# Autodesk Inventor assembly: naswietlarka uv
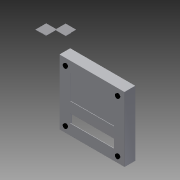
[picture p0: Inventor's stored thumbnail of the model, 180x180]
Saved by Autodesk Inventor 2014 (Build 180170000, 170)
## iProperties
Created: 2013-08-20
Part Number: naswietlarka uv
Document SubType Name: Assembly
Designer: Kisieel
Author: Kisieel
## Documents named in this file (23)
- D:\szkola\synergia\Naswietlarka\naswietlarka uv.iam
- D:\szkola\synergia\Naswietlarka\szyba.ipt
- D:\szkola\synergia\Naswietlarka\kątownik 1.ipt
- D:\szkola\synergia\Naswietlarka\kątownik 2.ipt
- D:\szkola\synergia\Naswietlarka\kątownik 3.ipt
- D:\szkola\synergia\Naswietlarka\blacha1.ipt
- D:\szkola\synergia\Naswietlarka\blacha2.ipt
- D:\szkola\synergia\Naswietlarka\kątownik_mały1.ipt
- D:\szkola\synergia\Naswietlarka\kątownik_mały2.ipt
- D:\szkola\synergia\Naswietlarka\kątownik_mały3.ipt
- D:\szkola\synergia\Naswietlarka\nóżka.ipt
- D:\szkola\synergia\Naswietlarka\świetlówka.ipt
- D:\szkola\synergia\Naswietlarka\uchwytG5.ipt
- D:\szkola\synergia\Naswietlarka\uchwytG5_MIR.ipt
- D:\szkola\synergia\Naswietlarka\Część5.ipt
- D:\szkola\synergia\Naswietlarka\wozek.ipt
- D:\szkola\synergia\Naswietlarka\podpora.ipt
- D:\szkola\synergia\Naswietlarka\kątownik_bloczek.ipt
- D:\szkola\synergia\Naswietlarka\poprzeczka.ipt
- D:\szkola\synergia\Naswietlarka\bloczek.ipt
- D:\szkola\synergia\Naswietlarka\sworzeń.ipt
- D:\szkola\synergia\Naswietlarka\zawias.ipt
- D:\szkola\synergia\Naswietlarka\zawias2.ipt
## Components (40 placed, 22 different names)
1. szyba:1 — Zestawiający:2, Równoległy:1, Zestawiający:3, Równoległy:2, Zestawiający:4, Zestawiający:6, Zestawiający:22
2. kątownik 1:1 — Zestawiający:2, Równoległy:1, Równoległy:3, Zestawiający:7, Równoległy:7, Równoległy:8, Zestawiający:10, Zestawiający:16, Zestawiający:24, Równoległy:14, Zestawiający:27, Styczny:2, Zestawiający:29, Styczny:5, Równoległy:19, Równoległy:21
3. kątownik 1:2 — Zestawiający:3, Równoległy:2, Równoległy:3, Równoległy:4, Równoległy:5, Zestawiający:5, Równoległy:6, Zestawiający:11, Zestawiający:15, Zestawiający:20, Zestawiający:23, Równoległy:13, Zestawiający:28, Styczny:4, Styczny:8, Zestawiający:33
4. kątownik 2:1 — Zestawiający:4, Równoległy:4, Równoległy:5, Zestawiający:8, Zestawiający:14, Równoległy:9, Styczny:1, Styczny:3, Zestawiający:72, Zestawiający:74
5. kątownik 3:1 — Zestawiający:5, Zestawiający:6, Równoległy:6, Zestawiający:9, Zestawiający:18, Zestawiający:25, Zestawiający:58, Zestawiający:62
6. kątownik 2:2 — Zestawiający:7, Równoległy:7, Równoległy:8, Zestawiający:26, Styczny:6, Zestawiający:30, Styczny:7, Zestawiający:32, Zestawiający:34
7. blacha1:1 — Zestawiający:8, Zestawiający:9, Zestawiający:10, Zestawiający:61, Zestawiający:73, Zestawiający:76
8. blacha2:1 — Zestawiający:11, Zestawiający:33, Zestawiający:34
9. kątownik_mały1:1 — Zestawiający:14, Równoległy:9, Zestawiający:15, Równoległy:10, Zestawiający:17
10. kątownik_mały2:1 — Zestawiający:16, Równoległy:10, Zestawiający:17, Równoległy:11, Zestawiający:19
11. kątownik_mały1:2 — Zestawiający:18, Równoległy:11, Zestawiający:19, Równoległy:12, Zestawiający:21, Zestawiający:22
12. kątownik_mały2:2 — Zestawiający:20, Równoległy:12, Zestawiający:21
13. kątownik_mały3:1 — Zestawiający:23, Równoległy:13, Zestawiający:26
14. kątownik_mały3:2 — Zestawiający:24, Równoległy:14, Zestawiający:25
15. nóżka:1 — Zestawiający:27, Styczny:1, Styczny:2, Zestawiający:31
16. nóżka:2 — Zestawiający:28, Styczny:3, Styczny:4
17. nóżka:3 — Zestawiający:30, Styczny:7, Styczny:8
18. nóżka:4 — Zestawiający:29, Styczny:5, Styczny:6
19. Część5:1 — Zestawiający:52, Zestawiający:53, Zestawiający:58, Symetria:1
20. wozek:1 — Zestawiający:52, Zestawiający:53, Zestawiający:57, Równoległy:15, Równoległy:16
21. Część5:2 — Zestawiający:61, Zestawiający:62, Zestawiający:69, Symetria:1
22. wozek:2 — Zestawiający:63, Równoległy:17, Zestawiający:64, Zestawiający:69, Zestawiający:78
23. podpora:1 — Zestawiający:57, Równoległy:15, Równoległy:16, Zestawiający:70, Równoległy:20, Zestawiający:71
24. podpora:2 — Zestawiający:63, Równoległy:17, Zestawiający:64, Zestawiający:65, Zestawiający:66, Równoległy:18, Zestawiający:77, Równoległy:22
25. kątownik_bloczek:1 — Zestawiający:72, Zestawiający:73, Zestawiający:75, Symetria:2, Zestawiający:79, Obrotowe:1
26. kątownik_bloczek:2 — Zestawiający:74, Zestawiający:75, Zestawiający:76, Symetria:2, Zestawiający:81
27. poprzeczka:1 — Zestawiający:77, Równoległy:22, Zestawiający:78
28. bloczek:1 — Zestawiający:80, Zestawiający:81
29. sworzeń:1 — Zestawiający:79, Obrotowe:1, Zestawiający:80
30. zawias:1
31. zawias2:1
32. świetlówka:1 — Zestawiający:35, Zestawiający:36, Zestawiający:37, Zestawiający:38, Kąt:2, Kąt:3
33. uchwytG5:1 — Zestawiający:35, Zestawiający:38, Kąt:1, Kąt:3, Równoległy:18
34. uchwytG5_MIR:1 — Zestawiający:36, Zestawiający:37, Kąt:1, Kąt:2
35. świetlówka:2
36. uchwytG5:2
37. uchwytG5_MIR:2
38. świetlówka:3
39. uchwytG5:3 — Zestawiający:65, Zestawiający:66
40. uchwytG5_MIR:3 — Zestawiający:70, Równoległy:20, Zestawiający:71
## Component patterns: (3 elements, first: świetlówka:1 + uchwytG5:1 + uchwytG5_MIR:1)
## Relationships (95: Mate 59, Flush 22, Tangent 8, Angle 3, Symmetry 2, RevoluteJoint 1)
- Zestawiający:2 [Mate]: szyba:1 ↔ kątownik 1:1
- Równoległy:1 [Flush]: szyba:1 ↔ kątownik 1:1
- Zestawiający:3 [Mate]: szyba:1 ↔ kątownik 1:2
- Równoległy:2 [Flush]: szyba:1 ↔ kątownik 1:2
- Równoległy:3 [Flush]: kątownik 1:1 ↔ kątownik 1:2
- Zestawiający:4 [Mate]: szyba:1 ↔ kątownik 2:1
- Równoległy:4 [Flush]: kątownik 1:2 ↔ kątownik 2:1
- Równoległy:5 [Flush]: kątownik 1:2 ↔ kątownik 2:1
- Zestawiający:5 [Mate]: kątownik 1:2 ↔ kątownik 3:1
- Zestawiający:6 [Mate]: szyba:1 ↔ kątownik 3:1
- Równoległy:6 [Flush]: kątownik 1:2 ↔ kątownik 3:1
- Zestawiający:7 [Mate]: kątownik 1:1 ↔ kątownik 2:2
- Równoległy:7 [Flush]: kątownik 1:1 ↔ kątownik 2:2
- Równoległy:8 [Flush]: kątownik 1:1 ↔ kątownik 2:2
- Zestawiający:8 [Mate]: kątownik 2:1 ↔ blacha1:1
- Zestawiający:9 [Mate] (5 mm): kątownik 3:1 ↔ blacha1:1
- Zestawiający:10 [Mate] (5 mm): kątownik 1:1 ↔ blacha1:1
- Zestawiający:11 [Mate] (44 mm): kątownik 1:2 ↔ blacha2:1
- Zestawiający:14 [Mate]: kątownik 2:1 ↔ kątownik_mały1:1
- Równoległy:9 [Flush] (10 mm): kątownik 2:1 ↔ kątownik_mały1:1
- Zestawiający:15 [Mate]: kątownik 1:2 ↔ kątownik_mały1:1
- Zestawiający:16 [Mate]: kątownik 1:1 ↔ kątownik_mały2:1
- Równoległy:10 [Flush]: kątownik_mały1:1 ↔ kątownik_mały2:1
- Zestawiający:17 [Mate]: kątownik_mały1:1 ↔ kątownik_mały2:1
- Zestawiający:18 [Mate]: kątownik 3:1 ↔ kątownik_mały1:2
- Równoległy:11 [Flush]: kątownik_mały2:1 ↔ kątownik_mały1:2
- Zestawiający:19 [Mate]: kątownik_mały2:1 ↔ kątownik_mały1:2
- Zestawiający:20 [Mate]: kątownik 1:2 ↔ kątownik_mały2:2
- Równoległy:12 [Flush]: kątownik_mały1:2 ↔ kątownik_mały2:2
- Zestawiający:21 [Mate]: kątownik_mały1:2 ↔ kątownik_mały2:2
- Zestawiający:22 [Mate]: szyba:1 ↔ kątownik_mały1:2
- Zestawiający:23 [Mate]: kątownik 1:2 ↔ kątownik_mały3:1
- Równoległy:13 [Flush] (4 mm): kątownik 1:2 ↔ kątownik_mały3:1
- Zestawiający:24 [Mate]: kątownik 1:1 ↔ kątownik_mały3:2
- Równoległy:14 [Flush] (2 mm): kątownik 1:1 ↔ kątownik_mały3:2
- Zestawiający:25 [Mate]: kątownik 3:1 ↔ kątownik_mały3:2
- Zestawiający:26 [Mate]: kątownik 2:2 ↔ kątownik_mały3:1
- Zestawiający:27 [Mate]: kątownik 1:1 ↔ nóżka:1
- Styczny:1 [Tangent] (20 mm): kątownik 2:1 ↔ nóżka:1
- Styczny:2 [Tangent] (20 mm): kątownik 1:1 ↔ nóżka:1
- Zestawiający:28 [Mate]: kątownik 1:2 ↔ nóżka:2
- Styczny:3 [Tangent] (20 mm): kątownik 2:1 ↔ nóżka:2
- Styczny:4 [Tangent] (20 mm): kątownik 1:2 ↔ nóżka:2
- Zestawiający:29 [Mate]: kątownik 1:1 ↔ nóżka:4
- Styczny:5 [Tangent] (20 mm): kątownik 1:1 ↔ nóżka:4
- Styczny:6 [Tangent] (20 mm): kątownik 2:2 ↔ nóżka:4
- Zestawiający:30 [Mate]: kątownik 2:2 ↔ nóżka:3
- Styczny:7 [Tangent] (20 mm): kątownik 2:2 ↔ nóżka:3
- Styczny:8 [Tangent] (20 mm): kątownik 1:2 ↔ nóżka:3
- Zestawiający:31 [Mate]: nóżka:1
- Zestawiający:32 [Mate]: kątownik 2:2
- Zestawiający:33 [Mate]: kątownik 1:2 ↔ blacha2:1
- Zestawiający:34 [Mate]: kątownik 2:2 ↔ blacha2:1
- Zestawiający:35 [Mate]: świetlówka:1 ↔ uchwytG5:1
- Zestawiający:36 [Mate]: świetlówka:1 ↔ uchwytG5_MIR:1
- Zestawiający:37 [Mate]: świetlówka:1 ↔ uchwytG5_MIR:1
- Zestawiający:38 [Mate]: świetlówka:1 ↔ uchwytG5:1
- Kąt:1 [Angle] (180 deg): uchwytG5:1 ↔ uchwytG5_MIR:1
- [Mate]: Część5:2 ↔ wozek:2
- Kąt:2 [Angle] (0 deg): świetlówka:1 ↔ uchwytG5_MIR:1
- Kąt:3 [Angle] (0 deg): świetlówka:1 ↔ uchwytG5:1
- Zestawiający:52 [Mate]: Część5:1 ↔ wozek:1
- Zestawiający:53 [Mate]: Część5:1 ↔ wozek:1
- Zestawiający:57 [Mate]: wozek:1 ↔ podpora:1
- Równoległy:15 [Flush]: wozek:1 ↔ podpora:1
- Równoległy:16 [Flush] (-3 mm): wozek:1 ↔ podpora:1
- Zestawiający:58 [Mate] (2 mm): kątownik 3:1 ↔ Część5:1
- Zestawiający:61 [Mate]: blacha1:1 ↔ Część5:2
- Zestawiający:62 [Mate] (2 mm): kątownik 3:1 ↔ Część5:2
- Zestawiający:63 [Mate]: wozek:2 ↔ podpora:2
- Równoległy:17 [Flush]: wozek:2 ↔ podpora:2
- Zestawiający:64 [Mate] (3 mm): wozek:2 ↔ podpora:2
- Zestawiający:65 [Mate] (1 mm): podpora:2 ↔ uchwytG5:3
- Zestawiający:66 [Mate]: podpora:2 ↔ uchwytG5:3
- Równoległy:18 [Flush]: podpora:2 ↔ uchwytG5:1
- Równoległy:19 [Flush] (150 mm): kątownik 1:1
- Zestawiający:69 [Mate]: Część5:2 ↔ wozek:2
- Zestawiający:70 [Mate]: podpora:1 ↔ uchwytG5_MIR:3
- Równoległy:20 [Flush]: podpora:1 ↔ uchwytG5_MIR:3
- Zestawiający:71 [Mate] (1 mm): podpora:1 ↔ uchwytG5_MIR:3
- Symetria:1 [Symmetry]: Część5:1 ↔ Część5:2
- Zestawiający:72 [Mate]: kątownik 2:1 ↔ kątownik_bloczek:1
- Zestawiający:73 [Mate]: blacha1:1 ↔ kątownik_bloczek:1
- Zestawiający:74 [Mate]: kątownik 2:1 ↔ kątownik_bloczek:2
- Zestawiający:75 [Mate] (20 mm): kątownik_bloczek:1 ↔ kątownik_bloczek:2
- Zestawiający:76 [Mate]: blacha1:1 ↔ kątownik_bloczek:2
- Równoległy:21 [Flush] (150 mm): kątownik 1:1
- Symetria:2 [Symmetry]: kątownik_bloczek:1 ↔ kątownik_bloczek:2
- Zestawiający:77 [Mate]: podpora:2 ↔ poprzeczka:1
- Równoległy:22 [Flush]: podpora:2 ↔ poprzeczka:1
- Zestawiający:78 [Mate]: wozek:2 ↔ poprzeczka:1
- Zestawiający:79 [Mate]: kątownik_bloczek:1 ↔ sworzeń:1
- Obrotowe:1 [RevoluteJoint] (-8 mm): kątownik_bloczek:1 ↔ sworzeń:1
- Zestawiający:80 [Mate]: bloczek:1 ↔ sworzeń:1
- Zestawiający:81 [Mate] (2 mm): kątownik_bloczek:2 ↔ bloczek:1
## Named parameters: d67_d65 = 0 mm
